# Autodesk Inventor assembly: MagnetAssembly
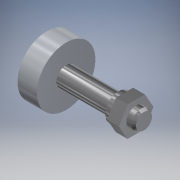
[picture p0: Inventor's stored thumbnail of the model, 180x180]
Saved by Autodesk Inventor 2017 (Build 210142000, 142)
## iProperties
Created: 2016-12-31
Part Number: MagnetAssembly
Document SubType Name: Assembly
Designer: umr
Author: umr
## Documents named in this file (4)
- D:\SeniorProject\Models2\HeadTools\MagnetAssembly.iam
- D:\SeniorProject\Models2\HeadTools\15mm x 5mm x 5mm Ring Magnet.ipt
- D:\SeniorProject\Models2\HeadTools\M5 Locknut.ipt
- D:\SeniorProject\Models2\HeadTools\M5 Screw_25mm.ipt
## Components (3 placed, 3 different names)
1. 15mm x 5mm x 5mm Ring Magnet:1 — Mate:1, Mate:3
2. M5 Locknut:1 — Mate:2, Flush:1
3. M5 Screw_25mm:1 — Mate:1, Mate:2, Flush:1, Mate:3
## Relationships (4: Mate 3, Flush 1)
- Mate:1: 15mm x 5mm x 5mm Ring Magnet:1 ↔ M5 Screw_25mm:1
- Mate:2: M5 Locknut:1 ↔ M5 Screw_25mm:1
- Flush:1 (2 mm): M5 Locknut:1 ↔ M5 Screw_25mm:1
- Mate:3: 15mm x 5mm x 5mm Ring Magnet:1 ↔ M5 Screw_25mm:1
